# Autodesk Inventor assembly: ThinBody
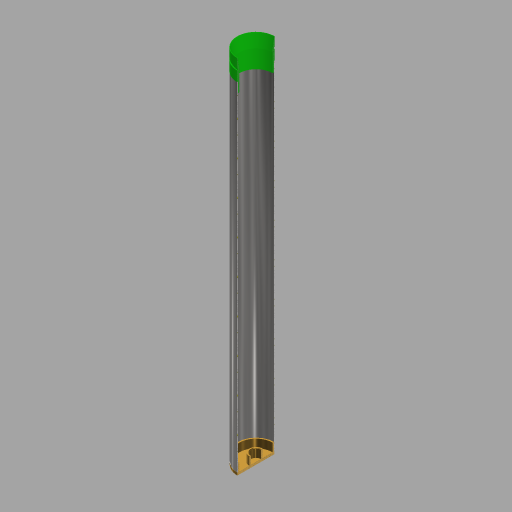
[picture p0: Inventor's stored thumbnail of the model, 512x512]
Saved by Autodesk Inventor 2024 (Build 280153020, 153B)
## iProperties
Created: 2023-09-25
Part Number: ThinBody
Document SubType Name: Assembly
Designer: schanen
Author: schanen
## Documents named in this file (4)
- C:\Users\schanen\Documents\Inventor\he4inserts\ThinBody.iam
- C:\Users\schanen\Documents\Inventor\he4inserts\BodyCylinderThin.ipt
- C:\Users\schanen\Documents\Inventor\he4inserts\CapCenterThin.ipt
- C:\Users\schanen\Documents\Inventor\he4inserts\CapConeThin.ipt
## Components (3 placed, 3 different names)
1. CapConeThin:1 — Mate:5
2. CapCenterThin:1 — Mate:1, Mate:2
3. BodyCylinderThin:1 — Mate:1, Mate:2, Mate:3, Mate:5
## Relationships (5: Mate 5)
- Mate:1: CapCenterThin:1 ↔ BodyCylinderThin:1
- Mate:2: CapCenterThin:1 ↔ BodyCylinderThin:1
- Mate:3: BodyCylinderThin:1
- [Mate]: CapConeThin:1 ↔ BodyCylinderThin:1
- Mate:5: CapConeThin:1 ↔ BodyCylinderThin:1
